# Autodesk Inventor assembly: Stiftleiste_Male_90_Gruppe
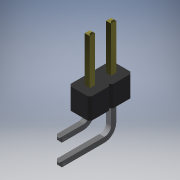
[picture p0: Inventor's stored thumbnail of the model, 180x180]
Saved by Autodesk Inventor 2017 SP1 (Build 210196100, 196)
## iProperties
Part Number: Stiftleiste_Male_90_Gruppe
Material: Generisch
Document SubType Name: Assembly
Designer: Alex
Author: Alex
## Documents named in this file (3)
- E:\Users\Alex\Documents\Inventor\Bauelemente\Buchsen_Stecker\Stiftleiste\Män\90_grad\Stiftleiste_Male_90_Gruppe.iam
- E:\Users\Alex\Documents\Inventor\Bauelemente\Buchsen_Stecker\Stiftleiste\Män\90_grad\Stiftleiste_Male_90_1.ipt
- E:\Users\Alex\Documents\Inventor\Bauelemente\Buchsen_Stecker\Stiftleiste\Män\90_grad\Stiftleiste_Male_90_2.ipt
## Components (2 placed, 2 different names)
1. Stiftleiste_Male_90_1:1 — Passend:1, Fluchtend:1, Fluchtend:2
2. Stiftleiste_Male_90_2:1 — Passend:1, Fluchtend:1, Fluchtend:2
## Relationships (3: Flush 2, Mate 1)
- Passend:1 [Mate]: Stiftleiste_Male_90_1:1 ↔ Stiftleiste_Male_90_2:1
- Fluchtend:1 [Flush]: Stiftleiste_Male_90_1:1 ↔ Stiftleiste_Male_90_2:1
- Fluchtend:2 [Flush]: Stiftleiste_Male_90_1:1 ↔ Stiftleiste_Male_90_2:1
